# Autodesk Inventor assembly: Tray
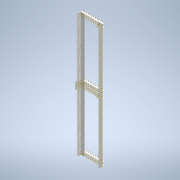
[picture p0: Inventor's stored thumbnail of the model, 180x180]
Saved by Autodesk Inventor 2020 (Build 240168000, 168)
## iProperties
Created: 2019-11-01
Part Number: Tray
Document SubType Name: Assembly
Designer: Alex Zaccardelli
Author: Alex Zaccardelli
## Documents named in this file (5)
- D:\DR4BTrayBot\Tray.iam
- D:\DR4BTrayBot\SIGBotsCADLibrary\Structure\C-Channel 2 x 12.ipt
- D:\DR4BTrayBot\SIGBotsCADLibrary\Structure\L-Channel 35 (aluminum).ipt
- D:\DR4BTrayBot\SIGBotsCADLibrary\Structure\Plate 2 x 3 (aluminum).ipt
- D:\DR4BTrayBot\SIGBotsCADLibrary\Structure\Plate 3 x 3 (aluminum).ipt
## Components (10 placed, 4 different names)
1. C-Channel 2 x 12:1 — Mate:1, Mate:2, Mate:3, Mate:4, Mate:5, Mate:6
2. L-Channel 35 (aluminum):1 — Mate:1, Mate:2, Mate:3, Mate:7, Mate:8, Mate:9, Mate:10, Mate:11, Mate:12, Flush:1
3. L-Channel 35 (aluminum):2 — Mate:4, Mate:5, Mate:6
4. C-Channel 2 x 12:2 — Mate:7, Mate:8, Mate:9
5. Plate 2 x 3 (aluminum):1 — Mate:10, Mate:11, Mate:12, Mate:25
6. C-Channel 2 x 12:3
7. L-Channel 35 (aluminum):3 — Mate:22, Mate:23, Mate:24, Flush:1
8. L-Channel 35 (aluminum):4
9. C-Channel 2 x 12:4
10. Plate 3 x 4:1 — Mate:22, Mate:23, Mate:24, Mate:25
## Relationships (26: Mate 25, Flush 1)
- Mate:1: C-Channel 2 x 12:1 ↔ L-Channel 35 (aluminum):1
- Mate:2: C-Channel 2 x 12:1 ↔ L-Channel 35 (aluminum):1
- Mate:3: C-Channel 2 x 12:1 ↔ L-Channel 35 (aluminum):1
- Mate:4: C-Channel 2 x 12:1 ↔ L-Channel 35 (aluminum):2
- Mate:5: C-Channel 2 x 12:1 ↔ L-Channel 35 (aluminum):2
- Mate:6: C-Channel 2 x 12:1 ↔ L-Channel 35 (aluminum):2
- Mate:7: L-Channel 35 (aluminum):1 ↔ C-Channel 2 x 12:2
- Mate:8: L-Channel 35 (aluminum):1 ↔ C-Channel 2 x 12:2
- Mate:9: L-Channel 35 (aluminum):1 ↔ C-Channel 2 x 12:2
- Mate:10: L-Channel 35 (aluminum):1 ↔ Plate 2 x 3 (aluminum):1
- Mate:11: L-Channel 35 (aluminum):1 ↔ Plate 2 x 3 (aluminum):1
- Mate:12: L-Channel 35 (aluminum):1 ↔ Plate 2 x 3 (aluminum):1
- [Mate]: C-Channel 2 x 12:3 ↔ L-Channel 35 (aluminum):3
- [Mate]: C-Channel 2 x 12:3 ↔ L-Channel 35 (aluminum):3
- [Mate]: C-Channel 2 x 12:3 ↔ L-Channel 35 (aluminum):3
- [Mate]: C-Channel 2 x 12:3 ↔ L-Channel 35 (aluminum):4
- [Mate]: C-Channel 2 x 12:3 ↔ L-Channel 35 (aluminum):4
- [Mate]: C-Channel 2 x 12:3 ↔ L-Channel 35 (aluminum):4
- [Mate]: L-Channel 35 (aluminum):3 ↔ C-Channel 2 x 12:4
- [Mate]: L-Channel 35 (aluminum):3 ↔ C-Channel 2 x 12:4
- [Mate]: L-Channel 35 (aluminum):3 ↔ C-Channel 2 x 12:4
- Mate:22: L-Channel 35 (aluminum):3 ↔ Plate 3 x 4:1
- Mate:23: L-Channel 35 (aluminum):3 ↔ Plate 3 x 4:1
- Mate:24: L-Channel 35 (aluminum):3 ↔ Plate 3 x 4:1
- Mate:25: Plate 2 x 3 (aluminum):1 ↔ Plate 3 x 4:1
- Flush:1: L-Channel 35 (aluminum):1 ↔ L-Channel 35 (aluminum):3
## Named parameters: d12_d3 = 0 mm, d13_d4 = 0 mm, d14_d5 = 0 mm, d15_d6 = 0 mm, d16_d7 = 0 mm, d17_d8 = 0 mm, d18_d0 = 0 mm, d19_d1 = 0 mm, d20_d2 = 0 mm
